# Autodesk Inventor assembly: LEG
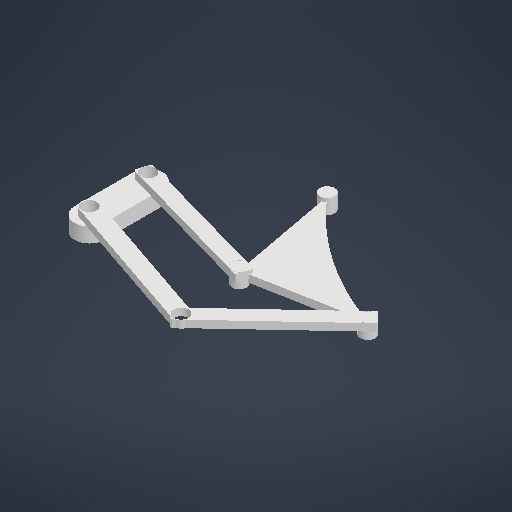
[picture p0: Inventor's stored thumbnail of the model, 512x512]
Saved by Autodesk Inventor 2027 (Build 310192060, 192F)
## iProperties
Created: 2026-08-01
Part Number: LEG
Document SubType Name: Assembly
Designer: User
Author: User
## Documents named in this file (5)
- G:\Github\Hot_dog\Hardware\Leg_concept\LEG.iam
- G:\Github\Hot_dog\Hardware\Leg_concept\Knee.ipt
- G:\Github\Hot_dog\Hardware\Leg_concept\foot.ipt
- G:\Github\Hot_dog\Hardware\Leg_concept\base.ipt
- G:\Github\Hot_dog\Hardware\Leg_concept\tibia.ipt
## Components (5 placed, 4 different names)
1. Knee:1 — Obrotowe:1, Obrotowe:2
2. foot:1 — Obrotowe:1, Obrotowe:6
3. foot:2 — Obrotowe:2, Obrotowe:4
4. base:1 — Obrotowe:4, Obrotowe:5
5. tibia:1 — Obrotowe:5, Obrotowe:6
## Relationships (5: RevoluteJoint 5)
- Obrotowe:1 [RevoluteJoint]: Knee:1 ↔ foot:1
- Obrotowe:2 [RevoluteJoint]: Knee:1 ↔ foot:2
- Obrotowe:4 [RevoluteJoint]: foot:2 ↔ base:1
- Obrotowe:5 [RevoluteJoint]: base:1 ↔ tibia:1
- Obrotowe:6 [RevoluteJoint]: foot:1 ↔ tibia:1
